# Autodesk Inventor assembly: Main Assembly
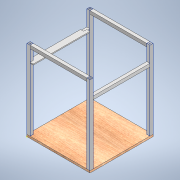
[picture p0: Inventor's stored thumbnail of the model, 180x180]
Saved by Autodesk Inventor 2020 (Build 240168000, 168)
## iProperties
Created: 2020-03-15
Part Number: Main Assembly
Document SubType Name: Assembly
Designer: Peter
Author: Peter
## Documents named in this file (7)
- C:\Users\Peter\Documents\Development\paragon-printer\Main Assembly.iam
- C:\Users\Peter\Documents\Development\paragon-printer\Stock\Base.ipt
- C:\Users\Peter\Documents\Development\paragon-printer\Stock\Tower.ipt
- C:\Users\Peter\Documents\Development\paragon-printer\Stock\X Cross Piece.ipt
- C:\Users\Peter\Documents\Development\paragon-printer\Stock\Y Cross Piece.ipt
- C:\Users\Peter\Documents\Development\paragon-printer\Stock\Top Sheet Metal Left.ipt
- C:\Users\Peter\Documents\Development\paragon-printer\Paragon Printer Parameters.xlsx
## Components (10 placed, 5 different names)
1. Base:1 — Mate:1, Mate:2, Mate:3, Mate:4, Mate:5, Flush:15
2. Tower:1 — Flush:3, Mate:4, Flush:6, Mate:12
3. Tower:2 — Flush:2, Flush:3, Mate:1, Mate:5, Flush:4, Flush:8, Mate:7
4. Tower:3 — Flush:1, Flush:2, Mate:3, Flush:4, Flush:5, Flush:7, Mate:6, Mate:9, Flush:10
5. Tower:4 — Flush:1, Mate:2, Flush:5, Flush:6, Mate:8, Flush:13, Mate:11
6. X Cross Piece:1 — Flush:7, Mate:6
7. X Cross Piece:2 — Flush:8, Mate:7
8. Y Cross Piece:1 — Mate:8, Flush:13, Flush:14, Mate:10
9. Y Cross Piece:2 — Mate:9, Flush:10, Flush:14, Flush:15
10. Top Sheet Metal Left:1 — Mate:10, Mate:11, Mate:12
## Relationships (24: Flush 12, Mate 12)
- Flush:1: Tower:3 ↔ Tower:4
- Flush:2: Tower:2 ↔ Tower:3
- Flush:3: Tower:1 ↔ Tower:2
- Mate:1: Base:1 ↔ Tower:2
- Mate:2: Base:1 ↔ Tower:4
- Mate:3: Base:1 ↔ Tower:3
- Mate:4: Base:1 ↔ Tower:1
- Mate:5: Base:1 ↔ Tower:2
- Flush:4: Tower:2 ↔ Tower:3
- Flush:5: Tower:3 ↔ Tower:4
- Flush:6: Tower:1 ↔ Tower:4
- Flush:7: Tower:3 ↔ X Cross Piece:1
- Mate:6: Tower:3 ↔ X Cross Piece:1
- Flush:8: Tower:2 ↔ X Cross Piece:2
- Mate:7: Tower:2 ↔ X Cross Piece:2
- Mate:8: Tower:4 ↔ Y Cross Piece:1
- Mate:9: Tower:3 ↔ Y Cross Piece:2
- Flush:10: Tower:3 ↔ Y Cross Piece:2
- Flush:13: Tower:4 ↔ Y Cross Piece:1
- Flush:14: Y Cross Piece:1 ↔ Y Cross Piece:2
- Flush:15 (-400 mm): Base:1 ↔ Y Cross Piece:2
- Mate:10: Y Cross Piece:1 ↔ Top Sheet Metal Left:1
- Mate:11: Tower:4 ↔ Top Sheet Metal Left:1
- Mate:12: Tower:1 ↔ Top Sheet Metal Left:1
## Named parameters: base_x_dim = 400 mm, base_y_dim = 400 mm, base_thickness = 12.7 mm, twenty = 20 mm, tower_height = 500 mm, extrusion_dim = 20 mm, ceiling_height = 400 mm, top_sheet_thickness = 6.35 mm, ceiling_width = 40 mm
